# Autodesk Inventor assembly: Pick_&_Place_Nozzle_Assembly
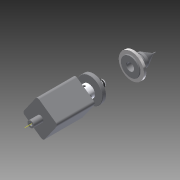
[picture p0: Inventor's stored thumbnail of the model, 180x180]
Saved by Autodesk Inventor 2015 (Build 190159000, 159)
## iProperties
Created: 2015-01-06
Part Number: Pick_&_Place_Nozzle_Assembly
Document SubType Name: Assembly
Designer: ice
Author: ice
## Documents named in this file (8)
- C:\Users\ice\Documents\GitHub\PnP-Magnetic-Tool-Tip\Inventor\Pick_&_Place_Nozzle_Assembly_Nozzle_#2.iam
- C:\Users\ice\Documents\GitHub\PnP-Magnetic-Tool-Tip\Inventor\Extender.ipt
- C:\Users\ice\Documents\GitHub\PnP-Magnetic-Tool-Tip\Inventor\NEMA8.ipt
- C:\Users\ice\Documents\GitHub\PnP-Magnetic-Tool-Tip\Inventor\Magnet20x3x5.ipt
- C:\Users\ice\Documents\GitHub\PnP-Magnetic-Tool-Tip\Inventor\Rubber_Seal2.ipt
- C:\Users\ice\Documents\GitHub\PnP-Magnetic-Tool-Tip\Inventor\Nozzle#2.ipt
- C:\Users\ice\Documents\GitHub\PnP-Magnetic-Tool-Tip\Inventor\M10_Ring.ipt
- C:\Users\ice\Documents\GitHub\PnP-Magnetic-Tool-Tip\Inventor\Rubber_Seal1.ipt
## Components (8 placed, 7 different names)
1. Extender:1 — Mate:5, Mate:10, Mate:11, Mate:12, Mate:13, Mate:14, Mate:16
2. NEMA8:1 — Mate:5, Mate:14
3. Magnet20x3x5:1 — Mate:10, Mate:11, Flush:2
4. Rubber_Seal2:1 — Mate:12
5. Rubber_Seal2:2 — Mate:13
6. Nozzle#2:1 — Mate:15, Mate:16, Flush:2, Mate:17, Flush:3
7. M10_Ring:1 — Mate:15, Flush:3
8. Rubber_Seal1:1 — Mate:17
## Relationships (11: Mate 9, Flush 2)
- Mate:5: Extender:1 ↔ NEMA8:1
- Mate:10: Extender:1 ↔ Magnet20x3x5:1
- Mate:11: Extender:1 ↔ Magnet20x3x5:1
- Mate:12: Extender:1 ↔ Rubber_Seal2:1
- Mate:13: Extender:1 ↔ Rubber_Seal2:2
- Mate:14: Extender:1 ↔ NEMA8:1
- Mate:15: Nozzle#2:1 ↔ M10_Ring:1
- Mate:16: Extender:1 ↔ Nozzle#2:1
- Flush:2: Magnet20x3x5:1 ↔ Nozzle#2:1
- Mate:17: Nozzle#2:1 ↔ Rubber_Seal1:1
- Flush:3: Nozzle#2:1 ↔ M10_Ring:1
